# Autodesk Inventor assembly: Ensamblaje_final
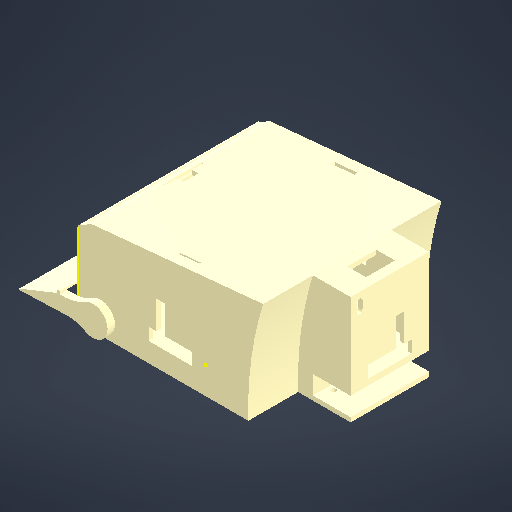
[picture p0: Inventor's stored thumbnail of the model, 512x512]
Saved by Autodesk Inventor 2026.2 (Build 302298010, 298A)
## iProperties
Created: 2026-05-09
Part Number: Ensamblaje_final
Document SubType Name: Assembly
Designer: migue
Author: migue
## Documents named in this file (4)
- C:\Users\migue\OneDrive\Documentos\2026-1\MPEI\PROYECTO MPEI\Ensamblaje_final.iam
- C:\Users\migue\OneDrive\Documentos\2026-1\MPEI\PROYECTO MPEI\cuchilla.ipt
- C:\Users\migue\OneDrive\Documentos\2026-1\MPEI\PROYECTO MPEI\Tapa V.2.ipt
- C:\Users\migue\OneDrive\Documentos\2026-1\MPEI\PROYECTO MPEI\Base V.2.ipt
## Components (3 placed, 3 different names)
1. cuchilla:1 — Insertar:1
2. Tapa V.2:1 — Rígido:1, Insertar:1
3. Base V.2:1 — Rígido:1
## Relationships (2: WeldJoint 1, Insert 1)
- Rígido:1 [WeldJoint]: Tapa V.2:1 ↔ Base V.2:1
- Insertar:1: cuchilla:1 ↔ Tapa V.2:1
